# Autodesk Inventor assembly: Clamping hub 6mm round shortened clamp
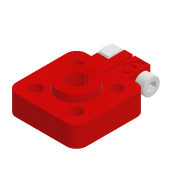
[picture p0: Inventor's stored thumbnail of the model, 180x180]
Saved by Autodesk Inventor 2020 (Build 240168000, 168)
## iProperties
Created: 2019-12-30
Part Number: Clamping hub 6mm round shortened clamp
Document SubType Name: Assembly
Designer: ball
Author: ball
## Documents named in this file (4)
- C:\FTC\FTC8863CAD\2019 Robot\Generic Parts\Clamping hub 6mm round shortened clamp.iam
- C:\FTC\FTC8863CAD\2019 Robot\Generic Parts\clamping hub 6mm round nut wells shortened clamp.ipt
- C:\FTC\FTC8863CAD\StepLibraries\Nuts\6-32 NYLON-INSERT LOCKNUT.ipt
- C:\FTC\FTC8863CAD\StepLibraries\Screws\6-32x.500 SOCKET HEAD CAP SCREW.ipt
## Components (7 placed, 3 different names)
1. clamping hub 6mm round nut wells shortened clamp:1 — Mate:1, Mate:2, Angle:1, Mate:3, Mate:4, Angle:2, Mate:5, Mate:6, Angle:3, Mate:7, Mate:8, Angle:4, Mate:9, Mate:10, Angle:5, Mate:11, Mate:12
2. 6-32 NYLON-INSERT LOCKNUT:1 — Mate:1, Mate:2, Angle:1
3. 6-32 NYLON-INSERT LOCKNUT:2 — Mate:3, Mate:4, Angle:2
4. 6-32 NYLON-INSERT LOCKNUT:3 — Mate:9, Mate:10, Angle:5
5. 6-32 NYLON-INSERT LOCKNUT:4 — Mate:5, Mate:6, Angle:3
6. 6-32 NYLON-INSERT LOCKNUT:5 — Mate:7, Mate:8, Angle:4
7. 6-32x.500 SOCKET HEAD CAP SCREW:1 — Mate:11, Mate:12
## Relationships (17: Mate 12, Angle 5)
- Mate:1: clamping hub 6mm round nut wells shortened clamp:1 ↔ 6-32 NYLON-INSERT LOCKNUT:1
- Mate:2: clamping hub 6mm round nut wells shortened clamp:1 ↔ 6-32 NYLON-INSERT LOCKNUT:1
- Angle:1 (0 deg): clamping hub 6mm round nut wells shortened clamp:1 ↔ 6-32 NYLON-INSERT LOCKNUT:1
- Mate:3: clamping hub 6mm round nut wells shortened clamp:1 ↔ 6-32 NYLON-INSERT LOCKNUT:2
- Mate:4: clamping hub 6mm round nut wells shortened clamp:1 ↔ 6-32 NYLON-INSERT LOCKNUT:2
- Angle:2 (0 deg): clamping hub 6mm round nut wells shortened clamp:1 ↔ 6-32 NYLON-INSERT LOCKNUT:2
- Mate:5: clamping hub 6mm round nut wells shortened clamp:1 ↔ 6-32 NYLON-INSERT LOCKNUT:4
- Mate:6: clamping hub 6mm round nut wells shortened clamp:1 ↔ 6-32 NYLON-INSERT LOCKNUT:4
- Angle:3 (0 deg): clamping hub 6mm round nut wells shortened clamp:1 ↔ 6-32 NYLON-INSERT LOCKNUT:4
- Mate:7: clamping hub 6mm round nut wells shortened clamp:1 ↔ 6-32 NYLON-INSERT LOCKNUT:5
- Mate:8: clamping hub 6mm round nut wells shortened clamp:1 ↔ 6-32 NYLON-INSERT LOCKNUT:5
- Angle:4 (0 deg): clamping hub 6mm round nut wells shortened clamp:1 ↔ 6-32 NYLON-INSERT LOCKNUT:5
- Mate:9: clamping hub 6mm round nut wells shortened clamp:1 ↔ 6-32 NYLON-INSERT LOCKNUT:3
- Mate:10: clamping hub 6mm round nut wells shortened clamp:1 ↔ 6-32 NYLON-INSERT LOCKNUT:3
- Angle:5 (0 deg): clamping hub 6mm round nut wells shortened clamp:1 ↔ 6-32 NYLON-INSERT LOCKNUT:3
- Mate:11: clamping hub 6mm round nut wells shortened clamp:1 ↔ 6-32x.500 SOCKET HEAD CAP SCREW:1
- Mate:12: clamping hub 6mm round nut wells shortened clamp:1 ↔ 6-32x.500 SOCKET HEAD CAP SCREW:1
